# Autodesk Inventor assembly: ASY PRS 9700 outlet pipe
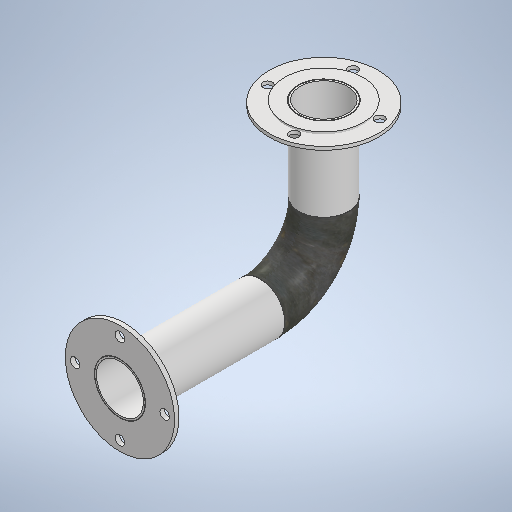
[picture p0: Inventor's stored thumbnail of the model, 512x512]
Saved by Autodesk Inventor 2026.2 (Build 302298000, 298)
## iProperties
Created: 2026-06-21
Part Number: ASY PRS 9700 outlet pipe
Document SubType Name: Assembly
Designer: admin
Author: admin
## Documents named in this file (7)
- C:\Users\admin\Documents\Inventor\PRS-Purovsk\ASY PRS 9700 outlet pipe.iam
- C:\Users\admin\Documents\Inventor\PRS-Purovsk\PRS 1633 charging blind flange_D1200 940.ipt
- C:\Users\admin\Documents\Inventor\PRS-Purovsk\PRS 9432 FDS free flange DN90_D1200 940.ipt
- C:\Users\admin\Documents\Inventor\PRS-Purovsk\PRS 9614 FDS tube 4_D1200 940.ipt
- C:\Users\admin\Documents\Inventor\PRS-Purovsk\PRS 9613 FDS tube 3_D1200 940.ipt
- C:\Users\admin\Documents\Inventor\PRS-Purovsk\cc\JIS B 2312 90 Deg Long Elbow Steel 80A x Sch 40.ipt
- C:\Users\admin\Documents\Inventor\PRS-Purovsk\PRS 9431 FDS flange DN90_D1200 940.ipt
## Components (6 placed, 6 different names)
1. PRS 1633 charging blind flange_D1200 940:1
2. PRS 9431 FDS flange DN90_D1200 940:1
3. PRS 9432 FDS free flange DN90_D1200 940:1
4. PRS 9614 FDS tube 4_D1200 940:1
5. PRS 9613 FDS tube 3_D1200 940:1
6. JIS B 2312 90 Deg Long Elbow Steel 80A x Sch 40:1
## Relationships (5: WeldJoint 4, RevoluteJoint 1)
- [RevoluteJoint]: PRS 9432 FDS free flange DN90_D1200 940:1 ↔ PRS 9614 FDS tube 4_D1200 940:1
- [WeldJoint]: PRS 1633 charging blind flange_D1200 940:1 ↔ PRS 9613 FDS tube 3_D1200 940:1
- [WeldJoint]: PRS 9614 FDS tube 4_D1200 940:1 ↔ JIS B 2312 90 Deg Long Elbow Steel 80A x Sch 40:1
- [WeldJoint]: PRS 9613 FDS tube 3_D1200 940:1 ↔ JIS B 2312 90 Deg Long Elbow Steel 80A x Sch 40:1
- [WeldJoint]: PRS 9431 FDS flange DN90_D1200 940:1 ↔ PRS 9432 FDS free flange DN90_D1200 940:1
